# Autodesk Inventor assembly: Assemblage_chassis_14_11
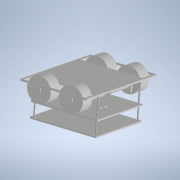
[picture p0: Inventor's stored thumbnail of the model, 180x180]
Saved by Autodesk Inventor 2020.1 (Build 241239000, 239)
## iProperties
Created: 2019-11-14
Part Number: Assemblage_chassis_14_11
Document SubType Name: Assembly
Designer: Admin
Author: Admin
## Documents named in this file (7)
- C:\Users\Admin\Desktop\Projet OrangeLab\CAO\Assemblage_chassis_14_11.iam
- C:\Users\Admin\Desktop\Projet OrangeLab\CAO\Chassis.ipt
- C:\Users\Admin\Desktop\Projet OrangeLab\CAO\Roue_moteur_MT.iam
- C:\Users\Admin\Desktop\Projet OrangeLab\CAO\Entretoises 80mm.ipt
- C:\Users\Admin\Desktop\Projet OrangeLab\CAO\Etage 1.ipt
- C:\Users\Admin\Desktop\Projet OrangeLab\CAO\Etage 2.ipt
- C:\Users\Admin\Desktop\Projet OrangeLab\CAO\Entretoises 50mm.ipt
## Components (15 placed, 6 different names)
1. Chassis:1 — Mate:1, Flush:1, Mate:2, Flush:2, Mate:3, Mate:4, Flush:3, Flush:4, Mate:5, Mate:6, Mate:7, Mate:8, Mate:9, Mate:10, Mate:11, Mate:12, Mate:13, Mate:14, Mate:15, Mate:16
2. Roue_moteur_MT:1 [sub-assembly] — Mate:4, Flush:3, Mate:7
3. Roue_moteur_MT:2 [sub-assembly] — Mate:3, Flush:4, Mate:8
4. Roue_moteur_MT:3 [sub-assembly] — Mate:1, Flush:1, Mate:6
5. Roue_moteur_MT:4 [sub-assembly] — Mate:2, Flush:2, Mate:5
6. Entretoises 80mm:1 — Mate:12, Mate:13
7. Entretoises 80mm:2 — Mate:9, Mate:14, Mate:18
8. Entretoises 80mm:3 — Mate:11, Mate:15, Mate:17, Mate:19
9. Entretoises 80mm:4 — Mate:10, Mate:16
10. Etage 1:1 — Mate:17, Mate:18, Mate:19, Mate:20, Mate:21, Mate:22, Mate:23, Mate:24, Mate:25, Mate:26, Mate:27
11. Etage 2:1 — Mate:28, Mate:29, Mate:30
12. Entretoises 50mm:1 — Mate:20, Mate:21
13. Entretoises 50mm:2 — Mate:24, Mate:25, Mate:29, Mate:30
14. Entretoises 50mm:3 — Mate:26, Mate:27
15. Entretoises 50mm:4 — Mate:22, Mate:23, Mate:28
## Relationships (34: Mate 30, Flush 4)
- Mate:1: Chassis:1 ↔ Roue_moteur_MT:3
- Flush:1: Chassis:1 ↔ Roue_moteur_MT:3
- Mate:2: Chassis:1 ↔ Roue_moteur_MT:4
- Flush:2: Chassis:1 ↔ Roue_moteur_MT:4
- Mate:3: Chassis:1 ↔ Roue_moteur_MT:2
- Mate:4: Chassis:1 ↔ Roue_moteur_MT:1
- Flush:3: Chassis:1 ↔ Roue_moteur_MT:1
- Flush:4: Chassis:1 ↔ Roue_moteur_MT:2
- Mate:5: Chassis:1 ↔ Roue_moteur_MT:4
- Mate:6: Chassis:1 ↔ Roue_moteur_MT:3
- Mate:7: Chassis:1 ↔ Roue_moteur_MT:1
- Mate:8: Chassis:1 ↔ Roue_moteur_MT:2
- Mate:9: Chassis:1 ↔ Entretoises 80mm:2
- Mate:10: Chassis:1 ↔ Entretoises 80mm:4
- Mate:11: Chassis:1 ↔ Entretoises 80mm:3
- Mate:12: Chassis:1 ↔ Entretoises 80mm:1
- Mate:13: Chassis:1 ↔ Entretoises 80mm:1
- Mate:14: Chassis:1 ↔ Entretoises 80mm:2
- Mate:15: Chassis:1 ↔ Entretoises 80mm:3
- Mate:16: Chassis:1 ↔ Entretoises 80mm:4
- Mate:17: Entretoises 80mm:3 ↔ Etage 1:1
- Mate:18: Entretoises 80mm:2 ↔ Etage 1:1
- Mate:19: Entretoises 80mm:3 ↔ Etage 1:1
- Mate:20: Etage 1:1 ↔ Entretoises 50mm:1
- Mate:21: Etage 1:1 ↔ Entretoises 50mm:1
- Mate:22: Etage 1:1 ↔ Entretoises 50mm:4
- Mate:23: Etage 1:1 ↔ Entretoises 50mm:4
- Mate:24: Etage 1:1 ↔ Entretoises 50mm:2
- Mate:25: Etage 1:1 ↔ Entretoises 50mm:2
- Mate:26: Etage 1:1 ↔ Entretoises 50mm:3
- Mate:27: Etage 1:1 ↔ Entretoises 50mm:3
- Mate:28: Etage 2:1 ↔ Entretoises 50mm:4
- Mate:29: Etage 2:1 ↔ Entretoises 50mm:2
- Mate:30: Etage 2:1 ↔ Entretoises 50mm:2
